# Autodesk Inventor assembly: FRA_MainAssembly_000
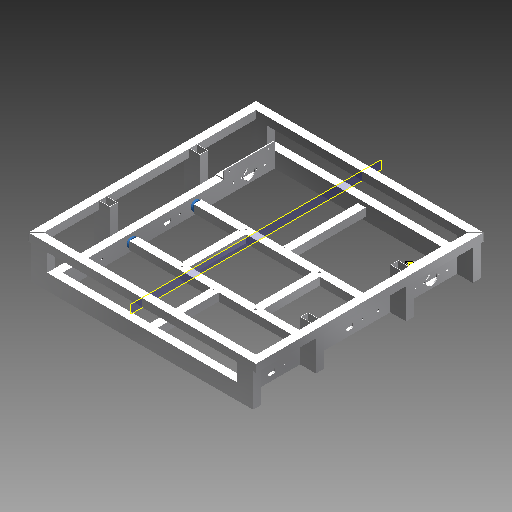
[picture p0: Inventor's stored thumbnail of the model, 512x512]
Saved by Autodesk Inventor 2018.3 (Build 223284000, 284)
## iProperties
Created: 2020-01-08
Part Number: FRA_MainAssembly_000
Document SubType Name: Assembly
Designer: user
Mass: 5217.89 g
Surface Area: 19836.3 cm^2
Volume: 1944.22 cm^3
Density: 2.6838 g/cm^3
Author: user
## Documents named in this file (15)
- C:\Users\22turnmaxw\Documents\GrabCAD\Infinite Recharge 2020\Build season\FRA_000_FullFrame.iam
- C:\Users\22turnmaxw\Documents\GrabCAD\Infinite Recharge 2020\Build season\FRA_001_MainRail.ipt
- C:\Users\22turnmaxw\Documents\GrabCAD\Infinite Recharge 2020\Build season\FRA_002_BackMainRail.ipt
- C:\Users\22turnmaxw\Documents\GrabCAD\Infinite Recharge 2020\Build season\FRA_004_TopSide.ipt
- C:\Users\22turnmaxw\Documents\GrabCAD\Infinite Recharge 2020\Build season\FRA_003_SideUpperSupport.ipt
- C:\Users\22turnmaxw\Documents\GrabCAD\Infinite Recharge 2020\Build season\FRA_005_CornerStandoffs.ipt
- C:\Users\22turnmaxw\Documents\GrabCAD\Infinite Recharge 2020\Build season\FRA_006_FrontMainRail.ipt
- C:\Users\22turnmaxw\Documents\GrabCAD\Infinite Recharge 2020\Build season\FRA_001_MainRail_MIR.ipt
- C:\Users\22turnmaxw\Documents\GrabCAD\Infinite Recharge 2020\Build season\FRA_009_1inCrossPlug.ipt
- C:\Users\22turnmaxw\Documents\GrabCAD\Infinite Recharge 2020\Build season\FRA_010_1inCrossSpacer.ipt
- C:\Users\22turnmaxw\Documents\GrabCAD\Infinite Recharge 2020\Build season\FRA_008_1inSideCenterSupports.ipt
- C:\Users\22turnmaxw\Documents\GrabCAD\Infinite Recharge 2020\Build season\FRA_014_AngleBracketGearbox.ipt
- C:\Users\22turnmaxw\Documents\GrabCAD\Infinite Recharge 2020\Build season\FRA_016_SmallTurntableSupports.ipt
- C:\Users\22turnmaxw\Documents\GrabCAD\Infinite Recharge 2020\Build season\FRA_017_BackCenterSupport.ipt
- C:\Users\22turnmaxw\Documents\GrabCAD\Infinite Recharge 2020\Build season\FRA_019_FrontCenterSupport.ipt
## Components (34 placed, 14 different names)
1. FRA_001_MainRail:1 — Mate:1, Flush:1, Mate:2, Mate:5, Mate:7, Mate:13, Flush:5, Mate:15, Mate:22, Mate:24, Mate:25, Flush:8, Mate:26, Mate:72, Mate:74, Mate:75, Mate:76, Mate:84, Mate:90, Mate:91, Mate:92, Mate:93
2. FRA_002_BackMainRail:1 — Mate:1, Flush:1, Mate:2, Mate:6, Mate:9, Flush:7, Mate:44
3. FRA_004_TopSide:1 — Mate:5, Mate:6, Mate:7, Mate:11, Flush:3, Mate:12, Mate:14, Flush:4, Mate:23, Mate:27, Mate:28, Flush:10, Mate:29, Symmetry:1
4. FRA_004_TopSide:2 — Mate:9, Flush:4, Mate:17, Mate:18, Mate:19, Mate:20, Mate:21, Symmetry:1
5. FRA_004_TopSide:3 — Mate:11, Flush:3, Mate:12, Mate:19, Flush:6, Mate:45
6. FRA_003_SideUpperSupport:1 — Flush:5, Mate:15, Mate:43, Flush:20
7. FRA_003_SideUpperSupport:2 — Mate:13, Mate:14, Mate:42, Mate:43, Flush:21
8. FRA_003_SideUpperSupport:3 — Mate:18, Mate:20, Flush:20
9. FRA_003_SideUpperSupport:4 — Mate:17, Mate:21, Flush:21
10. FRA_005_CornerStandoffs:1 — Mate:26, Mate:27, Flush:9
11. FRA_005_CornerStandoffs:2 — Flush:19, Mate:48, Mate:49
12. FRA_005_CornerStandoffs:3 — Flush:7, Mate:44, Mate:45
13. FRA_005_CornerStandoffs:4 — Mate:22, Mate:23, Flush:6, Mate:42
14. FRA_006_FrontMainRail:1 — Mate:24, Mate:25, Flush:8, Flush:9, Flush:19, Mate:48, Mate:70, Mate:96
15. FRA_004_TopSide:4 — Mate:28, Flush:10, Mate:29, Mate:49
16. FRA_001_MainRail_MIR:1 — Flush:22, Mate:80, Mate:81, Mate:87
17. FRA_009_1inCrossPlug:1
18. FRA_010_1inCrossSpacer:1 — Mate:72, Mate:76
19. FRA_009_1inCrossPlug:2
20. FRA_010_1inCrossSpacer:2
21. FRA_008_1inSideCenterSupports:1 — Mate:70, Flush:24, Flush:25, Mate:82, Mate:83, Flush:26, Flush:33, Flush:34
22. FRA_009_1inCrossPlug:3 — Mate:85, Flush:27
23. FRA_010_1inCrossSpacer:3 — Mate:74, Mate:75, Mate:86
24. FRA_009_1inCrossPlug:4 — Flush:28, Flush:29
25. FRA_010_1inCrossSpacer:4 — Mate:87
26. FRA_008_1inSideCenterSupports:2 — Flush:26, Mate:85, Mate:86, Flush:27, Flush:28, Flush:29, Mate:89, Flush:30, Flush:31, Flush:32
27. FRA_014_AngleBracketGearbox:1 — Mate:91, Mate:92, Mate:93
28. FRA_014_AngleBracketGearbox:2 — Flush:22, Mate:80, Mate:81
29. FRA_016_SmallTurntableSupports:1 — Flush:24, Mate:82, Mate:84, Mate:88, Flush:31, Flush:34
30. FRA_016_SmallTurntableSupports:2 — Flush:25, Mate:83, Mate:88, Flush:32, Flush:33
31. FRA_017_BackCenterSupport:1 — Mate:89, Flush:30, Mate:90, Mate:94, Mate:95, Flush:35, Flush:36, Flush:37
32. FRA_009_1inCrossPlug:5 — Mate:94, Mate:95, Flush:35
33. FRA_009_1inCrossPlug:6 — Mate:97, Mate:98, Flush:38
34. FRA_019_FrontCenterSupport:1 — Flush:36, Flush:37, Mate:96, Mate:97, Mate:98, Flush:38
## Relationships (97: Mate 68, Flush 28, Symmetry 1)
- Mate:1: FRA_001_MainRail:1 ↔ FRA_002_BackMainRail:1
- Flush:1: FRA_001_MainRail:1 ↔ FRA_002_BackMainRail:1
- Mate:2: FRA_001_MainRail:1 ↔ FRA_002_BackMainRail:1
- Mate:5 (34.925 mm): FRA_001_MainRail:1 ↔ FRA_004_TopSide:1
- Mate:6: FRA_002_BackMainRail:1 ↔ FRA_004_TopSide:1
- Mate:7 (57.15 mm): FRA_001_MainRail:1 ↔ FRA_004_TopSide:1
- Mate:9: FRA_002_BackMainRail:1 ↔ FRA_004_TopSide:2
- Mate:11: FRA_004_TopSide:1 ↔ FRA_004_TopSide:3
- Flush:3: FRA_004_TopSide:1 ↔ FRA_004_TopSide:3
- Mate:12: FRA_004_TopSide:1 ↔ FRA_004_TopSide:3
- Mate:13: FRA_001_MainRail:1 ↔ FRA_003_SideUpperSupport:2
- Mate:14: FRA_004_TopSide:1 ↔ FRA_003_SideUpperSupport:2
- Flush:4: FRA_004_TopSide:1 ↔ FRA_004_TopSide:2
- Flush:5: FRA_001_MainRail:1 ↔ FRA_003_SideUpperSupport:1
- Mate:15: FRA_001_MainRail:1 ↔ FRA_003_SideUpperSupport:1
- Mate:17: FRA_004_TopSide:2 ↔ FRA_003_SideUpperSupport:4
- Mate:18: FRA_004_TopSide:2 ↔ FRA_003_SideUpperSupport:3
- Mate:19: FRA_004_TopSide:2 ↔ FRA_004_TopSide:3
- Mate:20: FRA_004_TopSide:2 ↔ FRA_003_SideUpperSupport:3
- Mate:21: FRA_004_TopSide:2 ↔ FRA_003_SideUpperSupport:4
- Mate:22: FRA_001_MainRail:1 ↔ FRA_005_CornerStandoffs:4
- Mate:23: FRA_004_TopSide:1 ↔ FRA_005_CornerStandoffs:4
- Flush:6: FRA_004_TopSide:3 ↔ FRA_005_CornerStandoffs:4
- Flush:7: FRA_002_BackMainRail:1 ↔ FRA_005_CornerStandoffs:3
- Mate:24: FRA_001_MainRail:1 ↔ FRA_006_FrontMainRail:1
- Mate:25: FRA_001_MainRail:1 ↔ FRA_006_FrontMainRail:1
- Flush:8: FRA_001_MainRail:1 ↔ FRA_006_FrontMainRail:1
- Mate:26: FRA_001_MainRail:1 ↔ FRA_005_CornerStandoffs:1
- Mate:27: FRA_004_TopSide:1 ↔ FRA_005_CornerStandoffs:1
- Flush:9: FRA_005_CornerStandoffs:1 ↔ FRA_006_FrontMainRail:1
- Mate:28: FRA_004_TopSide:1 ↔ FRA_004_TopSide:4
- Flush:10: FRA_004_TopSide:1 ↔ FRA_004_TopSide:4
- Mate:29: FRA_004_TopSide:1 ↔ FRA_004_TopSide:4
- Mate:42 (190.5 mm): FRA_003_SideUpperSupport:2 ↔ FRA_005_CornerStandoffs:4
- Mate:43 (266.7 mm): FRA_003_SideUpperSupport:1 ↔ FRA_003_SideUpperSupport:2
- Mate:44 (-50.8 mm): FRA_002_BackMainRail:1 ↔ FRA_005_CornerStandoffs:3
- Mate:45: FRA_004_TopSide:3 ↔ FRA_005_CornerStandoffs:3
- Flush:19: FRA_005_CornerStandoffs:2 ↔ FRA_006_FrontMainRail:1
- Mate:48: FRA_005_CornerStandoffs:2 ↔ FRA_006_FrontMainRail:1
- Mate:49: FRA_005_CornerStandoffs:2 ↔ FRA_004_TopSide:4
- Symmetry:1: FRA_004_TopSide:1 ↔ FRA_004_TopSide:2
- Flush:20: FRA_003_SideUpperSupport:1 ↔ FRA_003_SideUpperSupport:3
- Flush:21: FRA_003_SideUpperSupport:2 ↔ FRA_003_SideUpperSupport:4
- [Mate]: FRA_009_1inCrossPlug:1 ↔ FRA_010_1inCrossSpacer:1
- [Mate]: FRA_009_1inCrossPlug:1 ↔ FRA_010_1inCrossSpacer:1
- [Mate]: FRA_009_1inCrossPlug:2 ↔ FRA_010_1inCrossSpacer:2
- [Mate]: FRA_009_1inCrossPlug:2 ↔ FRA_010_1inCrossSpacer:2
- [Mate]: FRA_009_1inCrossPlug:1 ↔ FRA_008_1inSideCenterSupports:1
- [Mate]: FRA_010_1inCrossSpacer:1 ↔ FRA_008_1inSideCenterSupports:1
- [Mate]: FRA_009_1inCrossPlug:1 ↔ FRA_008_1inSideCenterSupports:1
- [Mate]: FRA_009_1inCrossPlug:2 ↔ FRA_008_1inSideCenterSupports:1
- [Mate]: FRA_010_1inCrossSpacer:2 ↔ FRA_008_1inSideCenterSupports:1
- [Mate]: FRA_009_1inCrossPlug:2 ↔ FRA_008_1inSideCenterSupports:1
- [Mate]: FRA_009_1inCrossPlug:3 ↔ FRA_010_1inCrossSpacer:3
- [Mate]: FRA_009_1inCrossPlug:3 ↔ FRA_010_1inCrossSpacer:3
- [Mate]: FRA_009_1inCrossPlug:4 ↔ FRA_010_1inCrossSpacer:4
- [Mate]: FRA_009_1inCrossPlug:4 ↔ FRA_010_1inCrossSpacer:4
- Mate:70 (209.55 mm): FRA_006_FrontMainRail:1 ↔ FRA_008_1inSideCenterSupports:1
- Mate:72: FRA_001_MainRail:1 ↔ FRA_010_1inCrossSpacer:1
- Mate:74: FRA_001_MainRail:1 ↔ FRA_010_1inCrossSpacer:3
- Mate:75: FRA_001_MainRail:1 ↔ FRA_010_1inCrossSpacer:3
- Mate:76: FRA_001_MainRail:1 ↔ FRA_010_1inCrossSpacer:1
- Flush:22: FRA_001_MainRail_MIR:1 ↔ FRA_014_AngleBracketGearbox:2
- Mate:80: FRA_001_MainRail_MIR:1 ↔ FRA_014_AngleBracketGearbox:2
- Mate:81: FRA_001_MainRail_MIR:1 ↔ FRA_014_AngleBracketGearbox:2
- Flush:24: FRA_008_1inSideCenterSupports:1 ↔ FRA_016_SmallTurntableSupports:1
- Flush:25: FRA_008_1inSideCenterSupports:1 ↔ FRA_016_SmallTurntableSupports:2
- Mate:82: FRA_008_1inSideCenterSupports:1 ↔ FRA_016_SmallTurntableSupports:1
- Mate:83: FRA_008_1inSideCenterSupports:1 ↔ FRA_016_SmallTurntableSupports:2
- Mate:84 (150.7998 mm): FRA_001_MainRail:1 ↔ FRA_016_SmallTurntableSupports:1
- Flush:26: FRA_008_1inSideCenterSupports:1 ↔ FRA_008_1inSideCenterSupports:2
- Mate:85: FRA_009_1inCrossPlug:3 ↔ FRA_008_1inSideCenterSupports:2
- Mate:86: FRA_010_1inCrossSpacer:3 ↔ FRA_008_1inSideCenterSupports:2
- Flush:27 (1.5875 mm): FRA_009_1inCrossPlug:3 ↔ FRA_008_1inSideCenterSupports:2
- Flush:28 (1.5875 mm): FRA_009_1inCrossPlug:4 ↔ FRA_008_1inSideCenterSupports:2
- Flush:29 (1.5875 mm): FRA_009_1inCrossPlug:4 ↔ FRA_008_1inSideCenterSupports:2
- Mate:87: FRA_001_MainRail_MIR:1 ↔ FRA_010_1inCrossSpacer:4
- Mate:88 (212.7504 mm): FRA_016_SmallTurntableSupports:1 ↔ FRA_016_SmallTurntableSupports:2
- Mate:89: FRA_008_1inSideCenterSupports:2 ↔ FRA_017_BackCenterSupport:1
- Flush:30: FRA_008_1inSideCenterSupports:2 ↔ FRA_017_BackCenterSupport:1
- Mate:90 (269.875 mm): FRA_001_MainRail:1 ↔ FRA_017_BackCenterSupport:1
- Flush:31: FRA_008_1inSideCenterSupports:2 ↔ FRA_016_SmallTurntableSupports:1
- Flush:32: FRA_008_1inSideCenterSupports:2 ↔ FRA_016_SmallTurntableSupports:2
- Flush:33: FRA_008_1inSideCenterSupports:1 ↔ FRA_016_SmallTurntableSupports:2
- Flush:34: FRA_008_1inSideCenterSupports:1 ↔ FRA_016_SmallTurntableSupports:1
- Mate:91: FRA_001_MainRail:1 ↔ FRA_014_AngleBracketGearbox:1
- Mate:92: FRA_001_MainRail:1 ↔ FRA_014_AngleBracketGearbox:1
- Mate:93: FRA_001_MainRail:1 ↔ FRA_014_AngleBracketGearbox:1
- Mate:94: FRA_017_BackCenterSupport:1 ↔ FRA_009_1inCrossPlug:5
- Mate:95: FRA_017_BackCenterSupport:1 ↔ FRA_009_1inCrossPlug:5
- Flush:35: FRA_017_BackCenterSupport:1 ↔ FRA_009_1inCrossPlug:5
- Flush:36: FRA_017_BackCenterSupport:1 ↔ FRA_019_FrontCenterSupport:1
- Flush:37: FRA_017_BackCenterSupport:1 ↔ FRA_019_FrontCenterSupport:1
- Mate:96: FRA_006_FrontMainRail:1 ↔ FRA_019_FrontCenterSupport:1
- Mate:97: FRA_009_1inCrossPlug:6 ↔ FRA_019_FrontCenterSupport:1
- Mate:98: FRA_009_1inCrossPlug:6 ↔ FRA_019_FrontCenterSupport:1
- Flush:38: FRA_009_1inCrossPlug:6 ↔ FRA_019_FrontCenterSupport:1
## Named parameters: d92_d58 = 0 mm, d93_d59 = 0 mm, d94_d60 = 0 mm, d95_d61 = 0 mm
